# Autodesk Inventor assembly: Assembly_Cube_Kinematic_KES400_VCA_Mirror_Holder
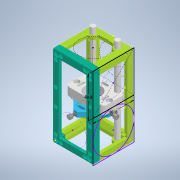
[picture p0: Inventor's stored thumbnail of the model, 180x180]
Saved by Autodesk Inventor 2022 (Build 260153000, 153)
## iProperties
Created: 2022-08-21
Part Number: Assembly_Cube_Kinematic_KES400_VCA_Mirror_Holder
Document SubType Name: Assembly
Designer: eda_b
Author: eda_b
## Documents named in this file (11)
- G:\My Drive\ASP - M.Sc. Photonics\Practical Modules\MODULE 4 - Master Thesis\2.Experiments\Modules\11.Reference_Mirror_Module\Reference_Mirror_with_KES400_VCA_Module\Assembly_Cube_Kinematic_KES400_VCA_Mirror_Holder.iam
- G:\My Drive\ASP - M.Sc. Photonics\Practical Modules\MODULE 4 - Master Thesis\2.Experiments\Modules\2.Base_Cube\Base_Cube_3DP\Base_Cube_3DP_2x1\with RODS\10_Cube_2x1_v3.ipt
- G:\My Drive\ASP - M.Sc. Photonics\Practical Modules\MODULE 4 - Master Thesis\2.Experiments\Modules\2.Base_Cube\Base_Cube_3DP\Base_Cube_3DP_2x1\with RODS\10_Lid_2x1_v3.ipt
- G:\My Drive\ASP - M.Sc. Photonics\Practical Modules\MODULE 4 - Master Thesis\2.Experiments\Modules\11.Reference_Mirror_Module\Reference_Mirror_with_KES400_VCA_Module\00_Thorlabs_Rod_6mm.ipt
- G:\My Drive\ASP - M.Sc. Photonics\Practical Modules\MODULE 4 - Master Thesis\2.Experiments\Modules\11.Reference_Mirror_Module\Reference_Mirror_with_KES400_VCA_Module\20_Cube_Insert_Kinematic_M12_VCAmount_Base_Thorlabs_Cage_Smaller.ipt
- G:\My Drive\ASP - M.Sc. Photonics\Practical Modules\MODULE 4 - Master Thesis\2.Experiments\Modules\11.Reference_Mirror_Module\Reference_Mirror_with_KES400_VCA_Module\20_Cube_Insert_Kinematic_KES400_VCAmount__90_pro_v3_rod.ipt
- G:\My Drive\ASP - M.Sc. Photonics\Practical Modules\MODULE 4 - Master Thesis\2.Experiments\Modules\11.Reference_Mirror_Module\Reference_Mirror_with_KES400_VCA_Module\00_KES400.iam
- C:\Users\eda_b\OneDrive\Belgeler\Inventor\Content Center Files\R2022\en-US\DIN 912\DIN 912 - M3 x 0.5 x 10 x 8.75.ipt
- C:\Users\eda_b\OneDrive\Belgeler\Inventor\Content Center Files\R2022\en-US\DIN 912\DIN 912 - M1.4 x 0.3 x 5 x 4.25.ipt
- G:\My Drive\ASP - M.Sc. Photonics\Practical Modules\MODULE 4 - Master Thesis\2.Experiments\Modules\11.Reference_Mirror_Module\Reference_Mirror_with_KES400_VCA_Module\00_coverglass_18mm.ipt
- C:\Users\eda_b\OneDrive\Belgeler\Inventor\Content Center Files\R2022\en-US\DIN 912\DIN 912 - M3 x 0.5 x 6 x 4.75.ipt
## Components (17 placed, 10 different names)
1. 10_Cube_2x1_v3:1 — Rotational:1, Rotational:2, Cylindrical:1, Cylindrical:2, Rotational:9, Rotational:10, Rotational:11, Rotational:12
2. 10_Lid_2x1_v3:1 — Rotational:1, Rotational:2
3. 00_Thorlabs_Rod_6mm:1 — Cylindrical:1, Cylindrical:3
4. 00_Thorlabs_Rod_6mm:2 — Cylindrical:2, Cylindrical:4
5. 20_Cube_Insert_Kinematic_M12_VCAmount_Base_Thorlabs_Cage_Smaller:1 — Cylindrical:3, Cylindrical:4, Rotational:3, Rigid:1
6. 20_Cube_Insert_Kinematic_KES400_VCAmount__90_pro_v3_rod:1 — Rotational:3, Rigid:1, Rotational:4, Rotational:5, Rigid:2, Rigid:3
7. 00_KES400:1 [sub-assembly] — Rotational:4, Rotational:5, Rotational:6, Rotational:7, Rotational:8, Rigid:4
8. DIN 912 - replaced by DIN EN ISO 4762 M3 x 10:1 — Rigid:3
9. DIN 912 - replaced by DIN EN ISO 4762 M1.4 x 5:3 — Rotational:8
10. DIN 912 - replaced by DIN EN ISO 4762 M1.4 x 5:1 — Rotational:6
11. DIN 912 - replaced by DIN EN ISO 4762 M3 x 10:4 — Rigid:2
12. DIN 912 - replaced by DIN EN ISO 4762 M1.4 x 5:2 — Rotational:7
13. 00_coverglass_18mm:1 — Rigid:4
14. DIN 912 - replaced by DIN EN ISO 4762 M3 x 6:1 — Rotational:12
15. DIN 912 - replaced by DIN EN ISO 4762 M3 x 6:2 — Rotational:9
16. DIN 912 - replaced by DIN EN ISO 4762 M3 x 6:3 — Rotational:11
17. DIN 912 - replaced by DIN EN ISO 4762 M3 x 6:4 — Rotational:10
## Relationships (20: RevoluteJoint 12, CylindricalJoint 4, WeldJoint 4)
- Rotational:1 [RevoluteJoint]: 10_Cube_2x1_v3:1 ↔ 10_Lid_2x1_v3:1
- Rotational:2 [RevoluteJoint]: 10_Cube_2x1_v3:1 ↔ 10_Lid_2x1_v3:1
- Cylindrical:1: 10_Cube_2x1_v3:1 ↔ 00_Thorlabs_Rod_6mm:1
- Cylindrical:2: 10_Cube_2x1_v3:1 ↔ 00_Thorlabs_Rod_6mm:2
- Cylindrical:3: 00_Thorlabs_Rod_6mm:1 ↔ 20_Cube_Insert_Kinematic_M12_VCAmount_Base_Thorlabs_Cage_Smaller:1
- Cylindrical:4: 00_Thorlabs_Rod_6mm:2 ↔ 20_Cube_Insert_Kinematic_M12_VCAmount_Base_Thorlabs_Cage_Smaller:1
- Rotational:3 [RevoluteJoint]: 20_Cube_Insert_Kinematic_M12_VCAmount_Base_Thorlabs_Cage_Smaller:1 ↔ 20_Cube_Insert_Kinematic_KES400_VCAmount__90_pro_v3_rod:1
- Rigid:1 [WeldJoint]: 20_Cube_Insert_Kinematic_M12_VCAmount_Base_Thorlabs_Cage_Smaller:1 ↔ 20_Cube_Insert_Kinematic_KES400_VCAmount__90_pro_v3_rod:1
- Rotational:4 [RevoluteJoint]: 20_Cube_Insert_Kinematic_KES400_VCAmount__90_pro_v3_rod:1 ↔ 00_KES400:1
- Rotational:5 [RevoluteJoint]: 20_Cube_Insert_Kinematic_KES400_VCAmount__90_pro_v3_rod:1 ↔ 00_KES400:1
- Rigid:2 [WeldJoint]: 20_Cube_Insert_Kinematic_KES400_VCAmount__90_pro_v3_rod:1 ↔ DIN 912 - replaced by DIN EN ISO 4762 M3 x 10:4
- Rigid:3 [WeldJoint]: 20_Cube_Insert_Kinematic_KES400_VCAmount__90_pro_v3_rod:1 ↔ DIN 912 - replaced by DIN EN ISO 4762 M3 x 10:1
- Rotational:6 [RevoluteJoint]: 00_KES400:1 ↔ DIN 912 - replaced by DIN EN ISO 4762 M1.4 x 5:1
- Rotational:7 [RevoluteJoint]: 00_KES400:1 ↔ DIN 912 - replaced by DIN EN ISO 4762 M1.4 x 5:2
- Rotational:8 [RevoluteJoint]: 00_KES400:1 ↔ DIN 912 - replaced by DIN EN ISO 4762 M1.4 x 5:3
- Rigid:4 [WeldJoint] (1 mm): 00_KES400:1 ↔ 00_coverglass_18mm:1
- Rotational:9 [RevoluteJoint]: 10_Cube_2x1_v3:1 ↔ DIN 912 - replaced by DIN EN ISO 4762 M3 x 6:2
- Rotational:10 [RevoluteJoint]: 10_Cube_2x1_v3:1 ↔ DIN 912 - replaced by DIN EN ISO 4762 M3 x 6:4
- Rotational:11 [RevoluteJoint]: 10_Cube_2x1_v3:1 ↔ DIN 912 - replaced by DIN EN ISO 4762 M3 x 6:3
- Rotational:12 [RevoluteJoint]: 10_Cube_2x1_v3:1 ↔ DIN 912 - replaced by DIN EN ISO 4762 M3 x 6:1
